# Autodesk Inventor assembly: ASY NVPH-300 hopper
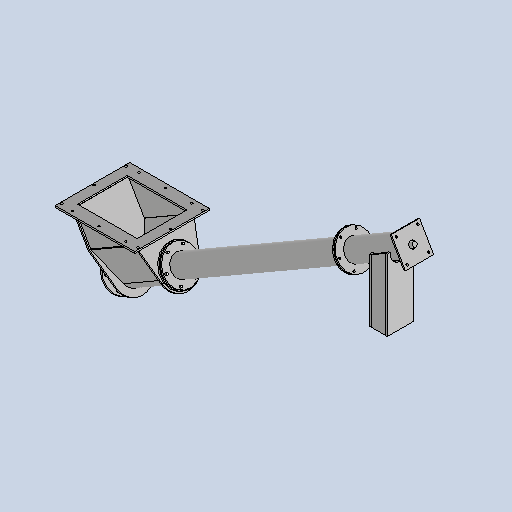
[picture p0: Inventor's stored thumbnail of the model, 512x512]
Saved by Autodesk Inventor 2025 (Build 290162010, 162A)
## iProperties
Created: 2024-12-19
Part Number: ASY NVPH-300 hopper
Document SubType Name: Assembly
Designer: admin
Author: admin
## Documents named in this file (14)
- C:\Users\admin\YandexDisk-badmisterfox\домашниий пк\Inventor\NDM-VOS_powder_hopper\ASY NVPH-300 hopper.iam
- C:\Users\admin\YandexDisk-badmisterfox\домашниий пк\Inventor\NDM-VOS_powder_hopper\NVPH-401 auger.ipt
- C:\Users\admin\YandexDisk-badmisterfox\домашниий пк\Inventor\NDM-VOS_powder_hopper\NVPH-301 back side.ipt
- C:\Users\admin\YandexDisk-badmisterfox\домашниий пк\Inventor\NDM-VOS_powder_hopper\NVPH-306 front side.ipt
- C:\Users\admin\YandexDisk-badmisterfox\домашниий пк\Inventor\NDM-VOS_powder_hopper\ASY NVPH-466 joint flange.iam
- C:\Users\admin\YandexDisk-badmisterfox\домашниий пк\Inventor\NDM-VOS_powder_hopper\NVPH-502 augur shaft.ipt
- C:\Users\admin\YandexDisk-badmisterfox\домашниий пк\Inventor\NDM-VOS_powder_hopper\ASY HPR 600 Feeder head.iam
- C:\Users\admin\YandexDisk-badmisterfox\домашниий пк\Inventor\NDM-VOS_powder_hopper\NVPH-406 second tube half.ipt
- C:\Users\admin\YandexDisk-badmisterfox\домашниий пк\Inventor\NDM-VOS_powder_hopper\NVPH-307 right side.ipt
- C:\Users\admin\YandexDisk-badmisterfox\домашниий пк\Inventor\NDM-VOS_powder_hopper\NVPH-316 main flange.ipt
- C:\Users\admin\YandexDisk-badmisterfox\домашниий пк\Inventor\NDM-VOS_powder_hopper\NVPH-418 revision cup.ipt
- C:\Users\admin\YandexDisk-badmisterfox\домашниий пк\Inventor\NDM-VOS_powder_hopper\NVPH-324 conductor.ipt
- C:\Users\admin\YandexDisk-badmisterfox\домашниий пк\Inventor\NDM-VOS_powder_hopper\NVPH-307 right side_MIR.ipt
- C:\Users\admin\YandexDisk-badmisterfox\домашниий пк\Inventor\NDM-VOS_powder_hopper\ASY HPR 340 hopper main tube.iam
## Components (16 placed, 13 different names)
1. NVPH-316 main flange:1 — Mate:4, Mate:5, Flush:1
2. NVPH-401 auger:1 — Rigid:12
3. NVPH-301 back side:1 — Mate:7
4. NVPH-306 front side:1
5. ASY NVPH-466 joint flange:1 [sub-assembly]
6. ASY NVPH-466 joint flange:2 [sub-assembly] — Flush:9
7. NVPH-502 augur shaft:1 — Rigid:12, Mate:6
8. ASY HPR 600 Feeder head:1 [sub-assembly] — Mate:6
9. NVPH-406 second tube half:1
10. NVPH-307 right side:1
11. NVPH-418 revision cup:1
12. NVPH-324 conductor:1
13. NVPH-324 conductor:2
14. Part1:1
15. ASY HPR 340 hopper main tube:1 [sub-assembly]
16. NVPH-307 right side:2
## Relationships (25: WeldJoint 10, Mate 7, CylindricalJoint 3, RevoluteJoint 2, Flush 2, Angle 1)
- [CylindricalJoint]: NVPH-401 auger:1 ↔ ASY HPR 340 hopper main tube:1
- [CylindricalJoint]: NVPH-301 back side:1 ↔ ASY HPR 340 hopper main tube:1
- [RevoluteJoint]: NVPH-301 back side:1 ↔ ASY NVPH-466 joint flange:1
- [CylindricalJoint]: NVPH-301 back side:1 ↔ NVPH-306 front side:1
- [RevoluteJoint]: NVPH-306 front side:1 ↔ ASY NVPH-466 joint flange:2
- [WeldJoint] (-2 mm): ASY HPR 600 Feeder head:1 ↔ ASY HPR 340 hopper main tube:1
- [WeldJoint]: NVPH-406 second tube half:1 ↔ NVPH-307 right side:1
- [WeldJoint]: NVPH-306 front side:1 ↔ NVPH-406 second tube half:1
- [Mate]: NVPH-301 back side:1 ↔ NVPH-406 second tube half:1
- [Mate]: NVPH-316 main flange:1 ↔ NVPH-306 front side:1
- [Angle] (-150 deg): NVPH-316 main flange:1 ↔ NVPH-406 second tube half:1
- [Mate]: NVPH-316 main flange:1 ↔ NVPH-306 front side:1
- [WeldJoint] (-50 mm): ASY NVPH-466 joint flange:1 ↔ NVPH-418 revision cup:1
- [WeldJoint]: ASY NVPH-466 joint flange:2 ↔ ASY HPR 340 hopper main tube:1
- [WeldJoint]: ASY HPR 600 Feeder head:1 ↔ ASY HPR 340 hopper main tube:1
- [WeldJoint]: NVPH-316 main flange:1 ↔ NVPH-324 conductor:2
- [WeldJoint]: NVPH-316 main flange:1 ↔ NVPH-324 conductor:1
- [WeldJoint]: NVPH-406 second tube half:1 ↔ Part1:1
- Mate:4: NVPH-316 main flange:1
- Mate:5: NVPH-316 main flange:1
- Flush:1: NVPH-316 main flange:1
- Rigid:12 [WeldJoint]: NVPH-401 auger:1 ↔ NVPH-502 augur shaft:1
- Mate:6 (10 mm): NVPH-502 augur shaft:1 ↔ ASY HPR 600 Feeder head:1
- Mate:7: NVPH-301 back side:1
- Flush:9: ASY NVPH-466 joint flange:2
